# Autodesk Inventor assembly: SansRotor
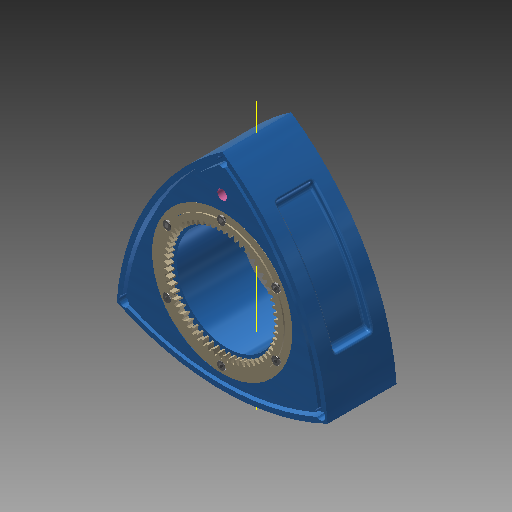
[picture p0: Inventor's stored thumbnail of the model, 512x512]
Saved by Autodesk Inventor 2019.4 (Build 234330000, 330)
## iProperties
Created: 2020-05-01
Part Number: SansRotor
Document SubType Name: Assembly
Designer: Gabriel
Author: Gabriel
## Documents named in this file (4)
- C:\Users\Gabriel\Desktop\Teme Gac\MotorWankel\SansRotor.iam
- C:\Users\Gabriel\Desktop\Teme Gac\MotorWankel\Rotor.ipt
- C:\Users\Gabriel\Desktop\Teme Gac\MotorWankel\Spur Gear21.ipt
- C:\Users\Gabriel\Desktop\Teme Gac\MotorWankel\SubAns-M4.iam
## Components (3 placed, 3 different names)
1. Rotor:1 — Mate:1, Mate:2, Mate:3, Mate:4, Mate:5, Angle:1
2. Spur Gear2:1 — Mate:4, Mate:5, Angle:1
3. SubAns-M4:1 [sub-assembly]
## Relationships (7: Mate 5, Angle 1, Insert 1)
- Mate:1: Rotor:1
- Mate:2: Rotor:1
- Mate:3: Rotor:1
- Mate:4: Rotor:1 ↔ Spur Gear2:1
- Mate:5: Rotor:1 ↔ Spur Gear2:1
- Angle:1 (0 deg): Rotor:1 ↔ Spur Gear2:1
- [Insert]: Spur Gear2:1 ↔ SubAns-M4:1
